# Autodesk Inventor assembly: 1in Actuator 1764
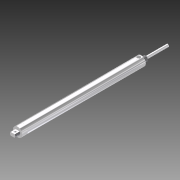
[picture p0: Inventor's stored thumbnail of the model, 180x180]
Saved by Autodesk Inventor 2011 (Build 150239000, 239)
## iProperties
Created: 2010-02-07
Part Number: 1in Actuator 1764
Document SubType Name: Assembly
Designer: jgehrig
Author: jgehrig
## Documents named in this file (5)
- R:\CAD Archives\Pneumatics\Actuators 1764\1in Actuator 1764\1in Actuator 1764.iam
- R:\CAD Archives\Pneumatics\Actuators 1764\1in Actuator 1764\1in Actuator Piston 1764.ipt
- R:\CAD Archives\Pneumatics\Actuators 1764\1in Actuator 1764\1in Actuator Housing 1764.ipt
- R:\CAD Archives\Pneumatics\Actuators 1764\1in Actuator 1764\1in Actuator Top Cap 1764.ipt
- R:\CAD Archives\Pneumatics\Actuators 1764\1in Actuator 1764\1in Actuator Bottom Cap 1764.ipt
## Components (4 placed, 4 different names)
1. 1in Actuator Housing 1764:1 — Insert:1, Insert:2, Mate:1
2. 1in Actuator Top Cap 1764:1 — Insert:2, Angle:1
3. 1in Actuator Piston 1764:1 — Mate:1
4. 1in Actuator Bottom Cap 1764:1 — Insert:1, Angle:1
## Relationships (4: Insert 2, Angle 1, Mate 1)
- Insert:1: 1in Actuator Housing 1764:1 ↔ 1in Actuator Bottom Cap 1764:1
- Insert:2: 1in Actuator Housing 1764:1 ↔ 1in Actuator Top Cap 1764:1
- Angle:1 (90 deg): 1in Actuator Top Cap 1764:1 ↔ 1in Actuator Bottom Cap 1764:1
- Mate:1: 1in Actuator Housing 1764:1 ↔ 1in Actuator Piston 1764:1
